# Autodesk Inventor assembly: Drinkmixer.Rohr- und Leitungsverläufe
(part 2 of 2)
- D:\Dropbox\My Dropbox\Dokumente\Aktuell\Drinkmixer\Drinkmixer\AIP\Rohr und Leitung\Drinkmixer.Rohr- und Leitungsverläufe.iam
- D:\Dropbox\My Dropbox\Dokumente\Aktuell\Drinkmixer\Drinkmixer\AIP\Rohr und Leitung\Verlauf01\Drinkmixer.Verlauf01.iam
## Components (1 placed, 1 different names)
1. Verlauf01 [sub-assembly]
